# Autodesk Inventor assembly: Chest
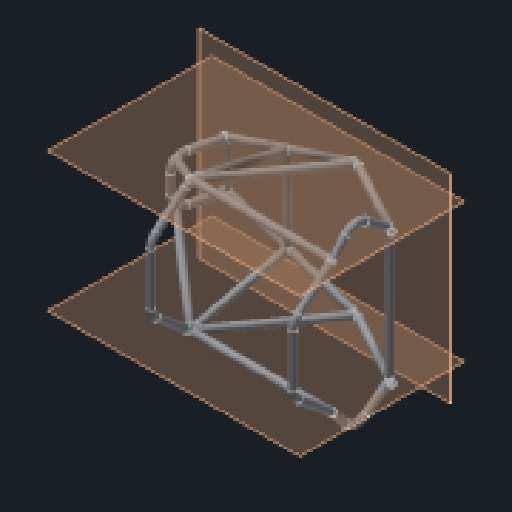
[picture p0: Inventor's stored thumbnail of the model, 512x512]
Saved by Autodesk Inventor 2025.2 (Build 292293000, 293)
## iProperties
Created: 2025-04-07
Part Number: Chest
Document SubType Name: Assembly
Designer: valer
Author: valer
## Documents named in this file (15)
- C:\Users\valer\Desktop\str1ker\cad\Chest.iam
- C:\Users\valer\Desktop\str1ker\cad\ChestBackTube.ipt
- C:\Users\valer\Desktop\str1ker\cad\ChestRightBottomTube.ipt
- C:\Users\valer\Desktop\str1ker\cad\ChestLeftBottomTube.ipt
- C:\Users\valer\Desktop\str1ker\cad\ChestTopRightTube.ipt
- C:\Users\valer\Desktop\str1ker\cad\ChestTopLeftTube.ipt
- C:\Users\valer\Desktop\str1ker\cad\ChestFrontTube.ipt
- C:\Users\valer\Desktop\str1ker\cad\ChestFrontBottomTube.ipt
- C:\Users\valer\Desktop\str1ker\cad\ChestMiddleTube.ipt
- C:\Users\valer\Desktop\str1ker\cad\ChestBackBottomTube.ipt
- C:\Users\valer\Desktop\str1ker\cad\ChestMiddleBackTube.ipt
- C:\Users\valer\Desktop\str1ker\cad\ChestBackRightTube.ipt
- C:\Users\valer\Desktop\str1ker\cad\ChestBackLeftTube.ipt
- C:\Users\valer\Desktop\str1ker\cad\ChestCrossLeftTube.ipt
- C:\Users\valer\Desktop\str1ker\cad\ChestCrossRightTube.ipt
## Components (14 placed, 14 different names)
1. ChestBackTube:1
2. ChestRightBottomTube:1
3. ChestLeftBottomTube:1
4. ChestTopRightTube:1
5. ChestTopLeftTube:1
6. ChestFrontTube:1
7. ChestFrontBottomTube:1
8. ChestMiddleTube:1
9. ChestBackBottomTube:1
10. ChestMiddleBackTube:1
11. ChestBackRightTube:1
12. ChestBackLeftTube:1
13. ChestCrossLeftTube:1
14. ChestCrossRightTube:1
## Relationships (3: Flush 3)
- Flush:1 (-9.5 mm)
- Flush:2 (184.5 mm)
- Flush:3 (-184.5 mm)
